# Autodesk Inventor assembly: spinning part
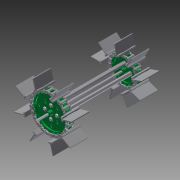
[picture p0: Inventor's stored thumbnail of the model, 180x180]
Saved by Autodesk Inventor 2014 SP1 (Build 180222100, 222)
## iProperties
Created: 2013-09-20
Part Number: spinning part
Document SubType Name: Assembly
Designer: Ryan
Author: Ryan
## Documents named in this file (9)
- C:\Users\Ryan\Desktop\pack and go\Workspaces\Workspace\toss up 1st A bot\toss up robot intake\spinning part.iam
- C:\Users\Ryan\Desktop\pack and go\Workspaces\Workspace\lib\Aperture VEX CAD Library\Sprockets\HS Sprockets\High strength Chain Link.ipt
- C:\Users\Ryan\Desktop\pack and go\Workspaces\Workspace\lib\Aperture VEX CAD Library\Tank Tread\flap-Link.ipt
- C:\Users\Ryan\Desktop\pack and go\Workspaces\Workspace\lib\Aperture VEX CAD Library\Tank Tread\flaps\Conveyor-Fin-Medium.ipt
- C:\Users\Ryan\Desktop\pack and go\Workspaces\Workspace\lib\Aperture VEX CAD Library\Standoffs\BEAM-6000.ipt
- C:\Users\Ryan\Desktop\pack and go\Workspaces\Workspace\lib\Aperture VEX CAD Library\Hardware\8-32\8-32_.375.ipt
- C:\Users\Ryan\Desktop\pack and go\Workspaces\Workspace\lib\Aperture VEX CAD Library\Shaft\9 inch Shaft.ipt
- C:\Users\Ryan\Desktop\pack and go\Workspaces\Workspace\lib\Aperture VEX CAD Library\Sprockets\green\High Strength 24-Tooth Sprocket.ipt
- C:\Users\Ryan\Desktop\pack and go\Workspaces\Workspace\lib\Aperture VEX CAD Library\Sprockets\green\High Strength 18-Tooth Sprocket.ipt
## Components (74 placed, 8 different names)
1. 9 inch Shaft:1 — Mate:31, Mate:32, Mate:46, Mate:47
2. High Strength 24-Tooth Sprocket:1 — Mate:31, Mate:32, Mate:33, Mate:35, Mate:36, Mate:37, Mate:38, Mate:39, Mate:41, Mate:42, Mate:43
3. High Strength 18-Tooth Sprocket:1 — Mate:44, Mate:45, Mate:46, Mate:47, Mate:48, Mate:49, Mate:50, Mate:51
4. High strength Chain Link:1 — Flush:1, Mate:35, Mate:36, Mate:37, Mate:40
5. High strength Chain Link:29 — Mate:39, Mate:40, Mate:41
6. Conveyor-Fin-Medium:1 — Mate:7, Flush:2, Mate:8
7. flap-Link:1 — Mate:5, Mate:7, Flush:2, Mate:8, Mate:38
8. High strength Chain Link:30
9. High strength Chain Link:31
10. Conveyor-Fin-Medium:15
11. flap-Link:15
12. High strength Chain Link:32
13. High strength Chain Link:33
14. Conveyor-Fin-Medium:16
15. flap-Link:16
16. High strength Chain Link:34
17. High strength Chain Link:35
18. Conveyor-Fin-Medium:17
19. flap-Link:17
20. High strength Chain Link:36
21. High strength Chain Link:37
22. Conveyor-Fin-Medium:18
23. flap-Link:18
24. High strength Chain Link:38
25. High strength Chain Link:39
26. Conveyor-Fin-Medium:19
27. flap-Link:19
28. High strength Chain Link:40
29. High strength Chain Link:41
30. Conveyor-Fin-Medium:20
31. flap-Link:20
32. High strength Chain Link:42
33. High strength Chain Link:43
34. Conveyor-Fin-Medium:21
35. flap-Link:21
36. 8-32_.375:2 — Mate:42, Mate:43
37. BEAM-6000:3 — Mate:30, Mate:33, Mate:44
38. 8-32_.375:1 — Mate:30, Mate:45, Mate:48
39. 8-32_.375:3
40. BEAM-6000:4
41. 8-32_.375:4
42. 8-32_.375:5
43. BEAM-6000:5
44. 8-32_.375:6
45. 8-32_.375:7
46. BEAM-6000:6
47. 8-32_.375:8
48. High strength Chain Link:17 — Flush:3, Mate:25, Mate:49, Mate:50, Mate:51
49. flap-Link:9 — Mate:52, Mate:25, Mate:26, Mate:27, Flush:28
50. Conveyor-Fin-Medium:9 — Mate:26, Mate:27, Flush:28
51. High strength Chain Link:44
52. flap-Link:22
53. Conveyor-Fin-Medium:22
54. High strength Chain Link:45
55. flap-Link:23
56. Conveyor-Fin-Medium:23
57. High strength Chain Link:46
58. flap-Link:24
59. Conveyor-Fin-Medium:24
60. High strength Chain Link:47
61. flap-Link:25
62. Conveyor-Fin-Medium:25
63. High strength Chain Link:48
64. flap-Link:26
65. Conveyor-Fin-Medium:26
66. High strength Chain Link:49
67. flap-Link:27
68. Conveyor-Fin-Medium:27
69. High strength Chain Link:50
70. flap-Link:28
71. Conveyor-Fin-Medium:28
72. High strength Chain Link:51
73. flap-Link:29
74. Conveyor-Fin-Medium:29
## Component patterns: (8 elements, first: High strength Chain Link:1 + High strength Chain Link:29 + Conveyor-Fin-Medium:1 + flap-Link:1), (4 elements, first: 8-32_.375:2 + BEAM-6000:3 + 8-32_.375:1), (9 elements, first: High strength Chain Link:17 + flap-Link:9 + Conveyor-Fin-Medium:9)
## Relationships (32: Mate 28, Flush 4)
- Flush:1 (4.0005 mm): High strength Chain Link:1
- Mate:5: flap-Link:1
- Mate:7: Conveyor-Fin-Medium:1 ↔ flap-Link:1
- Flush:2: Conveyor-Fin-Medium:1 ↔ flap-Link:1
- Mate:8: Conveyor-Fin-Medium:1 ↔ flap-Link:1
- Flush:3 (5.6007 mm): High strength Chain Link:17
- Mate:52: flap-Link:9
- Mate:25: High strength Chain Link:17 ↔ flap-Link:9
- Mate:26: flap-Link:9 ↔ Conveyor-Fin-Medium:9
- Mate:27: flap-Link:9 ↔ Conveyor-Fin-Medium:9
- Flush:28: flap-Link:9 ↔ Conveyor-Fin-Medium:9
- Mate:30: BEAM-6000:3 ↔ 8-32_.375:1
- Mate:31: 9 inch Shaft:1 ↔ High Strength 24-Tooth Sprocket:1
- Mate:32: 9 inch Shaft:1 ↔ High Strength 24-Tooth Sprocket:1
- Mate:33: High Strength 24-Tooth Sprocket:1 ↔ BEAM-6000:3
- Mate:35: High Strength 24-Tooth Sprocket:1 ↔ High strength Chain Link:1
- Mate:36: High Strength 24-Tooth Sprocket:1 ↔ High strength Chain Link:1
- Mate:37: High Strength 24-Tooth Sprocket:1 ↔ High strength Chain Link:1
- Mate:38: High Strength 24-Tooth Sprocket:1 ↔ flap-Link:1
- Mate:39: High Strength 24-Tooth Sprocket:1 ↔ High strength Chain Link:29
- Mate:40: High strength Chain Link:1 ↔ High strength Chain Link:29
- Mate:41: High Strength 24-Tooth Sprocket:1 ↔ High strength Chain Link:29
- Mate:42: High Strength 24-Tooth Sprocket:1 ↔ 8-32_.375:2
- Mate:43: High Strength 24-Tooth Sprocket:1 ↔ 8-32_.375:2
- Mate:44: High Strength 18-Tooth Sprocket:1 ↔ BEAM-6000:3
- Mate:45: High Strength 18-Tooth Sprocket:1 ↔ 8-32_.375:1
- Mate:46: 9 inch Shaft:1 ↔ High Strength 18-Tooth Sprocket:1
- Mate:47: 9 inch Shaft:1 ↔ High Strength 18-Tooth Sprocket:1
- Mate:48: High Strength 18-Tooth Sprocket:1 ↔ 8-32_.375:1
- Mate:49: High Strength 18-Tooth Sprocket:1 ↔ High strength Chain Link:17
- Mate:50: High Strength 18-Tooth Sprocket:1 ↔ High strength Chain Link:17
- Mate:51: High Strength 18-Tooth Sprocket:1 ↔ High strength Chain Link:17
